# Autodesk Inventor assembly: Falcon with Gearbox 2 stage_MIR
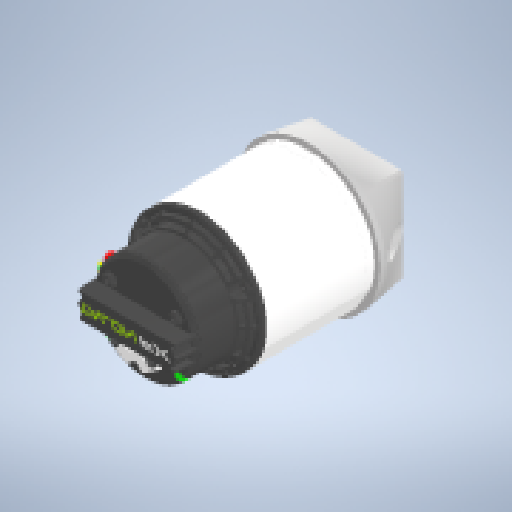
[picture p0: Inventor's stored thumbnail of the model, 512x512]
Saved by Autodesk Inventor 2023 (Build 270158000, 158)
## iProperties
Created: 2023-02-06
Part Number: Falcon with Gearbox 2 stage_MIR
Document SubType Name: Assembly
Designer: Gabriel - T3 CAD
Author: Gabriel - T3 CAD
## Documents named in this file (3)
- C:\Users\Gabriel - T3 CAD\Documents\GitHub\T3-CAD\Stock\Motors and Gearboxes\Falcon with Gearbox 2 stage_MIR.iam
- C:\Users\Gabriel - T3 CAD\Documents\GitHub\T3-CAD\Stock\Electronics\Falcon 500_MIR.ipt
- C:\Users\Gabriel - T3 CAD\Documents\GitHub\T3-CAD\Stock\Motors and Gearboxes\VersaPlanetary CIM Adapter (217-4018)_MIR.ipt
## Components (2 placed, 2 different names)
1. Falcon 500_MIR:1 — Rotational:2, Rotational:1
2. VersaPlanetary CIM Adapter (217-4018)_MIR:1 — Rotational:2, Rotational:1
## Relationships (2: RevoluteJoint 2)
- Rotational:2 [RevoluteJoint]: Falcon 500_MIR:1 ↔ VersaPlanetary CIM Adapter (217-4018)_MIR:1
- Rotational:1 [RevoluteJoint]: Falcon 500_MIR:1 ↔ VersaPlanetary CIM Adapter (217-4018)_MIR:1
